# Autodesk Inventor assembly: slideOut
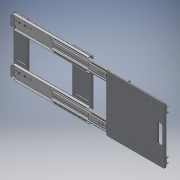
[picture p0: Inventor's stored thumbnail of the model, 180x180]
Saved by Autodesk Inventor 2016 (Build 200138000, 138)
## iProperties
Created: 2019-01-08
Part Number: slideOut
Document SubType Name: Assembly
Designer: harveylab
Author: harveylab
## Documents named in this file (5)
- C:\Users\harveylab\Documents\GitHub\mouseVR\Hardware\SlideOut\slideOut.iam
- C:\Users\harveylab\Documents\GitHub\mouseVR\Hardware\SlideOut\1102A640_BASE-MOUNT DRAWER SLIDE.ipt
- C:\Users\harveylab\Documents\GitHub\mouseVR\Hardware\SlideOut\vrRig_v08_breadboardToSlideMount.ipt
- C:\Users\harveylab\Documents\GitHub\mouseVR\Hardware\SlideOut\vrRig_v08_slideMountBottom.ipt
- C:\Users\harveylab\Documents\GitHub\mouseVR\Hardware\SlideOut\McM_92220A181_LOW-PROFILE ALLOY STEEL SOCKET HEAD CAP SCREW.ipt
## Components (12 placed, 4 different names)
1. 1102A640_BASE-MOUNT DRAWER SLIDE:1 — Insert:3, Mate:1, Insert:5, Insert:6, Insert:7, Insert:10, Insert:11
2. 1102A640_BASE-MOUNT DRAWER SLIDE:2 — Insert:1, Insert:2, Insert:4, Mate:2, Insert:8, Insert:9, Insert:12, Insert:13
3. vrRig_v08_breadboardToSlideMount:1 — Insert:4, Mate:1, Insert:5
4. vrRig_v08_slideMountBottom:1 — Insert:1, Insert:2, Insert:3, Mate:2
5. McM_92220A181_LOW-PROFILE ALLOY STEEL SOCKET HEAD CAP SCREW:1 — Insert:12
6. McM_92220A181_LOW-PROFILE ALLOY STEEL SOCKET HEAD CAP SCREW:2 — Insert:13
7. McM_92220A181_LOW-PROFILE ALLOY STEEL SOCKET HEAD CAP SCREW:3 — Insert:6
8. McM_92220A181_LOW-PROFILE ALLOY STEEL SOCKET HEAD CAP SCREW:4 — Insert:7
9. McM_92220A181_LOW-PROFILE ALLOY STEEL SOCKET HEAD CAP SCREW:5 — Insert:8
10. McM_92220A181_LOW-PROFILE ALLOY STEEL SOCKET HEAD CAP SCREW:6 — Insert:9
11. McM_92220A181_LOW-PROFILE ALLOY STEEL SOCKET HEAD CAP SCREW:7 — Insert:11
12. McM_92220A181_LOW-PROFILE ALLOY STEEL SOCKET HEAD CAP SCREW:8 — Insert:10
## Relationships (15: Insert 13, Mate 2)
- Insert:1: 1102A640_BASE-MOUNT DRAWER SLIDE:2 ↔ vrRig_v08_slideMountBottom:1
- Insert:2: 1102A640_BASE-MOUNT DRAWER SLIDE:2 ↔ vrRig_v08_slideMountBottom:1
- Insert:3: 1102A640_BASE-MOUNT DRAWER SLIDE:1 ↔ vrRig_v08_slideMountBottom:1
- Insert:4: 1102A640_BASE-MOUNT DRAWER SLIDE:2 ↔ vrRig_v08_breadboardToSlideMount:1
- Mate:1: 1102A640_BASE-MOUNT DRAWER SLIDE:1 ↔ vrRig_v08_breadboardToSlideMount:1
- Insert:5: 1102A640_BASE-MOUNT DRAWER SLIDE:1 ↔ vrRig_v08_breadboardToSlideMount:1
- Mate:2: 1102A640_BASE-MOUNT DRAWER SLIDE:2 ↔ vrRig_v08_slideMountBottom:1
- Insert:6: 1102A640_BASE-MOUNT DRAWER SLIDE:1 ↔ McM_92220A181_LOW-PROFILE ALLOY STEEL SOCKET HEAD CAP SCREW:3
- Insert:7: 1102A640_BASE-MOUNT DRAWER SLIDE:1 ↔ McM_92220A181_LOW-PROFILE ALLOY STEEL SOCKET HEAD CAP SCREW:4
- Insert:8: 1102A640_BASE-MOUNT DRAWER SLIDE:2 ↔ McM_92220A181_LOW-PROFILE ALLOY STEEL SOCKET HEAD CAP SCREW:5
- Insert:9: 1102A640_BASE-MOUNT DRAWER SLIDE:2 ↔ McM_92220A181_LOW-PROFILE ALLOY STEEL SOCKET HEAD CAP SCREW:6
- Insert:10: 1102A640_BASE-MOUNT DRAWER SLIDE:1 ↔ McM_92220A181_LOW-PROFILE ALLOY STEEL SOCKET HEAD CAP SCREW:8
- Insert:11: 1102A640_BASE-MOUNT DRAWER SLIDE:1 ↔ McM_92220A181_LOW-PROFILE ALLOY STEEL SOCKET HEAD CAP SCREW:7
- Insert:12: 1102A640_BASE-MOUNT DRAWER SLIDE:2 ↔ McM_92220A181_LOW-PROFILE ALLOY STEEL SOCKET HEAD CAP SCREW:1
- Insert:13: 1102A640_BASE-MOUNT DRAWER SLIDE:2 ↔ McM_92220A181_LOW-PROFILE ALLOY STEEL SOCKET HEAD CAP SCREW:2
